# Autodesk Inventor assembly: maze_version1
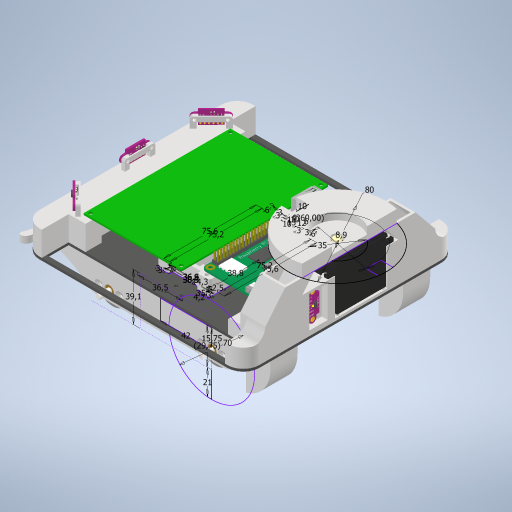
[picture p0: Inventor's stored thumbnail of the model, 512x512]
Saved by Autodesk Inventor 2023 (Build 270158000, 158)
## iProperties
Created: 2026-02-09
Part Number: maze_version1
Document SubType Name: Assembly
Designer: garin
Author: garin
## Documents named in this file (21)
- C:\Users\garin\OneDrive\Документы\maze\version1\maze_version1.iam
- C:\Users\garin\OneDrive\Документы\maze\version1\base.ipt
- C:\Users\garin\OneDrive\Документы\maze\version1\fast_battery.ipt
- C:\Users\garin\OneDrive\Документы\maze\version1\front_part_1.ipt
- C:\Users\garin\OneDrive\Документы\maze\version1\front_part_2.ipt
- C:\Users\garin\OneDrive\Документы\VL53L0X_TOF.ipt
- C:\Users\garin\OneDrive\Документы\maze\version1\fast_RGB.ipt
- C:\Users\garin\OneDrive\Документы\maze\version1\TCS34725 RGB sensor.ipt
- C:\Users\garin\OneDrive\Документы\maze\version1\end_cap.ipt
- C:\Users\garin\OneDrive\Документы\maze\version1\back_part.ipt
- C:\Users\garin\OneDrive\Документы\maze\version1\MG996R.ipt
- C:\Users\garin\OneDrive\Документы\maze\version1\raspberry_pi_5.ipt
- C:\Users\garin\OneDrive\Документы\maze\version1\board.ipt
- C:\Users\garin\OneDrive\Документы\maze\version1\motor_25_110RPM.ipt
- C:\Users\garin\OneDrive\Документы\maze\version1\circle.ipt
- C:\Users\garin\OneDrive\Документы\maze\version1\колёса.ipt
- C:\Users\garin\OneDrive\Документы\maze\version1\fast_motors_left.ipt
- C:\Users\garin\OneDrive\Документы\maze\version1\fast_motors_right.ipt
- C:\Users\garin\OneDrive\Документы\maze\version1\fast_akkum.ipt
- C:\Users\garin\OneDrive\Документы\maze\version1\fast_akkum2.ipt
- C:\Users\garin\OneDrive\Документы\maze\version1\system_extradition.ipt
## Components (27 placed, 20 different names)
1. base:1 — Заподлицо:1, Заподлицо:2, Заподлицо:3, Заподлицо:4, С поворотом:5, Заподлицо:6, С поворотом:15, С поворотом:18, С поворотом:19, Заподлицо:10, С поворотом:21, Заподлицо:11
2. fast_battery:1 — Заподлицо:1
3. front_part_1:1 — Заподлицо:2, С поворотом:6, Заподлицо:5, С поворотом:10, С поворотом:21
4. front_part_2:1 — Заподлицо:3, Заподлицо:4, С поворотом:6, С поворотом:7, С поворотом:8, С поворотом:11, С поворотом:14
5. fast_RGB:1 — С поворотом:5, С поворотом:9
6. VL53L0X_TOF:1 — С поворотом:7
7. VL53L0X_TOF:2 — С поворотом:8
8. TCS34725 RGB sensor:1 — С поворотом:9
9. end_cap:1 — Заподлицо:5
10. end_cap:2 — С поворотом:10
11. VL53L0X_TOF:3 — С поворотом:11
12. back_part:1 — Заподлицо:6, С поворотом:15, С поворотом:16, С поворотом:17, С поворотом:20
13. MG996R:1 — С поворотом:16, Заподлицо:7, Заподлицо:9
14. raspberry_pi_5:1 — С поворотом:17
15. board:1 — С поворотом:14
16. motor_25_110RPM:2
17. motor_25_110RPM:3
18. motor_25_110RPM:4
19. motor_25_110RPM:5
20. circle:1 — Заподлицо:7, Заподлицо:9, Заподлицо:12
21. колёса:1
22. fast_motors_left:1 — С поворотом:18
23. fast_motors_right:1 — С поворотом:19
24. VL53L0X_TOF:4 — С поворотом:20
25. fast_akkum:1 — Заподлицо:10
26. fast_akkum2:1 — Заподлицо:11
27. system_extradition:1 — Заподлицо:12
## Relationships (26: RevoluteJoint 15, Flush 11)
- Заподлицо:1 [Flush]: base:1 ↔ fast_battery:1
- Заподлицо:2 [Flush]: base:1 ↔ front_part_1:1
- Заподлицо:3 [Flush]: base:1 ↔ front_part_2:1
- Заподлицо:4 [Flush] (9 mm): base:1 ↔ front_part_2:1
- С поворотом:5 [RevoluteJoint]: base:1 ↔ fast_RGB:1
- С поворотом:6 [RevoluteJoint]: front_part_1:1 ↔ front_part_2:1
- С поворотом:7 [RevoluteJoint]: front_part_2:1 ↔ VL53L0X_TOF:1
- С поворотом:8 [RevoluteJoint]: front_part_2:1 ↔ VL53L0X_TOF:2
- С поворотом:9 [RevoluteJoint]: fast_RGB:1 ↔ TCS34725 RGB sensor:1
- Заподлицо:5 [Flush]: front_part_1:1 ↔ end_cap:1
- С поворотом:10 [RevoluteJoint]: front_part_1:1 ↔ end_cap:2
- С поворотом:11 [RevoluteJoint]: front_part_2:1 ↔ VL53L0X_TOF:3
- Заподлицо:6 [Flush]: base:1 ↔ back_part:1
- С поворотом:14 [RevoluteJoint]: front_part_2:1 ↔ board:1
- С поворотом:15 [RevoluteJoint]: base:1 ↔ back_part:1
- С поворотом:16 [RevoluteJoint]: back_part:1 ↔ MG996R:1
- С поворотом:17 [RevoluteJoint]: back_part:1 ↔ raspberry_pi_5:1
- Заподлицо:7 [Flush]: MG996R:1 ↔ circle:1
- Заподлицо:9 [Flush] (0.2 mm): MG996R:1 ↔ circle:1
- С поворотом:18 [RevoluteJoint]: base:1 ↔ fast_motors_left:1
- С поворотом:19 [RevoluteJoint]: base:1 ↔ fast_motors_right:1
- С поворотом:20 [RevoluteJoint]: back_part:1 ↔ VL53L0X_TOF:4
- Заподлицо:10 [Flush]: base:1 ↔ fast_akkum:1
- С поворотом:21 [RevoluteJoint]: base:1 ↔ front_part_1:1
- Заподлицо:11 [Flush]: base:1 ↔ fast_akkum2:1
- Заподлицо:12 [Flush]: circle:1 ↔ system_extradition:1
